# Autodesk Inventor assembly: paint platform assy2
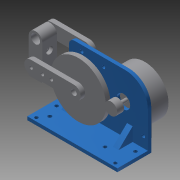
[picture p0: Inventor's stored thumbnail of the model, 180x180]
Saved by Autodesk Inventor 2013 SP2 (Build 170200200, 200)
## iProperties
Created: 2017-01-29
Part Number: paint platform assy2
Document SubType Name: Assembly
Designer: Herman de Vries
Author: Herman de Vries
## Documents named in this file (7)
- C:\Users\Herman de Vries\Dropbox\Projects\Inventor\PaintBot_3\paint platform assy2.iam
- C:\Users\Herman de Vries\Dropbox\Projects\Inventor\PaintBot_3\paint holder 2.ipt
- C:\Users\Herman de Vries\Dropbox\Projects\Inventor\PaintBot_3\stepper motor 1.ipt
- C:\Users\Herman de Vries\Dropbox\Projects\Inventor\PaintBot_3\gear.ipt
- C:\Users\Herman de Vries\Dropbox\Projects\Inventor\PaintBot_3\z axis arm1.ipt
- C:\Users\Herman de Vries\Dropbox\Projects\Inventor\PaintBot_3\z axis arm3.ipt
- C:\Users\Herman de Vries\Dropbox\Projects\Inventor\PaintBot_3\z axis arm2.ipt
## Components (6 placed, 6 different names)
1. paint holder 2:1 — Insert:1, Insert:8, Insert:9, Insert:10
2. stepper motor 1:1 — Insert:1, Insert:10
3. gear:1 — Insert:4, Insert:5, Insert:9
4. z axis arm1:1 — Insert:8, Mate:1
5. z axis arm3:1 — Mate:1, Insert:11
6. z axis arm2:1 — Insert:4, Insert:5, Insert:11
## Relationships (8: Insert 7, Mate 1)
- Insert:1: paint holder 2:1 ↔ stepper motor 1:1
- Insert:4: gear:1 ↔ z axis arm2:1
- Insert:5: gear:1 ↔ z axis arm2:1
- Insert:8: paint holder 2:1 ↔ z axis arm1:1
- Insert:9: paint holder 2:1 ↔ gear:1
- Insert:10: paint holder 2:1 ↔ stepper motor 1:1
- Mate:1: z axis arm1:1 ↔ z axis arm3:1
- Insert:11: z axis arm3:1 ↔ z axis arm2:1
